# Autodesk Inventor assembly: xy forearm
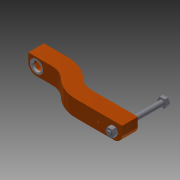
[picture p0: Inventor's stored thumbnail of the model, 180x180]
Saved by Autodesk Inventor 2013 (Build 170138000, 138)
## iProperties
Created: 2013-10-15
Part Number: xy forearm
Document SubType Name: Assembly
Designer: employee
Author: employee
## Documents named in this file (6)
- C:\Users\employee\Desktop\ConceptFORGE\ConceptFORGE\Wally\INVENTOR\xy forearm.iam
- C:\Users\employee\Desktop\ConceptFORGE\ConceptFORGE\Wally\INVENTOR\xy forearm.ipt
- C:\Users\employee\Desktop\ConceptFORGE\ConceptFORGE\Wally\INVENTOR\M3x16.ipt
- C:\Users\employee\Desktop\ConceptFORGE\ConceptFORGE\Wally\INVENTOR\6702.ipt
- C:\Users\employee\Desktop\ConceptFORGE\ConceptFORGE\Wally\INVENTOR\M8 nut.ipt
- C:\Users\employee\Desktop\ConceptFORGE\ConceptFORGE\Wally\INVENTOR\M8x85.ipt
## Components (6 placed, 5 different names)
1. xy forearm:1 — Insert:1, Mate:1, Mate:2, Mate:3, Insert:2, Insert:3, Mate:4
2. Forged Socket Head Cap Screw - Metric M3x0.5 x 16:1 — Mate:2, Mate:3
3. 6702:1 — Insert:1
4. 6702:2 — Insert:2
5. Hex Nut Metric M8 x 1.25:1 — Insert:3
6. M8x85 — Mate:1, Mate:4
## Relationships (7: Mate 4, Insert 3)
- Insert:1: xy forearm:1 ↔ 6702:1
- Mate:1: xy forearm:1 ↔ M8x85
- Mate:2 (5 mm): xy forearm:1 ↔ Forged Socket Head Cap Screw - Metric M3x0.5 x 16:1
- Mate:3: xy forearm:1 ↔ Forged Socket Head Cap Screw - Metric M3x0.5 x 16:1
- Insert:2: xy forearm:1 ↔ 6702:2
- Insert:3: xy forearm:1 ↔ Hex Nut Metric M8 x 1.25:1
- Mate:4 (51.5 mm): xy forearm:1 ↔ M8x85
